# Autodesk Inventor assembly: PrzeniesienieNapedu
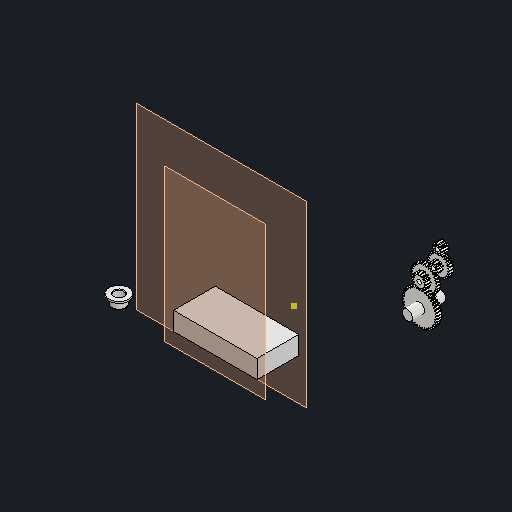
[picture p0: Inventor's stored thumbnail of the model, 512x512]
Saved by Autodesk Inventor 2023 (Build 270158000, 158)
## iProperties
Created: 2024-01-12
Part Number: PrzeniesienieNapedu
Document SubType Name: Assembly
Designer: Michał
Author: Michał
## Documents named in this file (6)
- D:\Projekty\Roboilo\Ser\3D\3D\V2\PrzeniesienieNapedu.iam
- D:\Projekty\Roboilo\Ser\3D\3D\PrzekladniaLewa\Design Accelerator\Przekładnie walcowe4.iam
- D:\Projekty\Roboilo\Ser\3D\3D\PrzekladniaLewa\Design Accelerator\Przekładnie walcowe3.iam
- D:\Projekty\Roboilo\Ser\3D\3D\PrzekladniaLewa\Design Accelerator\Przekładnie walcowe2.iam
- D:\Projekty\Roboilo\Ser\3D\3D\Lozysko GFM-0608-06.ipt
- D:\Projekty\Roboilo\Ser\3D\3D\V2\MocowanieLewejPrzekladni.ipt
## Components (5 placed, 3 different names)
1. Przekładnie walcowe:1 [sub-assembly] — Insert:2
2. Przekładnie walcowe:2 [sub-assembly] — Insert:1, Insert:2
3. Przekładnie walcowe:3 [sub-assembly] — Insert:1
4. Lozysko GFM-0608-06:1
5. MocowanieLewejPrzekladni:1
## Relationships (2: Insert 2)
- Insert:1: Przekładnie walcowe:2 ↔ Przekładnie walcowe:3
- Insert:2: Przekładnie walcowe:1 ↔ Przekładnie walcowe:2
